# Autodesk Inventor assembly: mg996r leg bottom middle
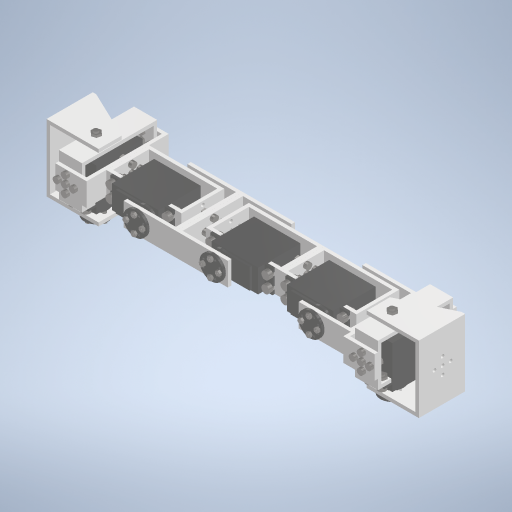
[picture p0: Inventor's stored thumbnail of the model, 512x512]
Saved by Autodesk Inventor 2023 (Build 270158000, 158)
## iProperties
Created: 2022-06-29
Part Number: mg996r leg bottom middle
Document SubType Name: Assembly
Designer: isamu
Author: isamu
## Documents named in this file (6)
- D:\personal_projects\robot\inventor\mg996r left leg bottom middle.iam
- D:\personal_projects\robot\inventor\mg996r 3mm middle base leg.iam
- D:\personal_projects\robot\inventor\mg996r 3mm foot.iam
- D:\personal_projects\robot\exports\frames\m3x8.ipt
- D:\personal_projects\robot\exports\frames\m3 nuts.ipt
- D:\personal_projects\robot\inventor\mg996r 3mm center frame.iam
## Components (23 placed, 5 different names)
1. mg996r 3mm middle base leg:1 [sub-assembly] — Mate:1, Mate:2, Mate:3, Insert:1, Insert:2, Insert:3, Insert:4, Insert:5, Mate:4, Mate:5, Mate:6, Insert:11, Insert:12, Insert:13, Insert:14, Insert:15
2. mg996r 3mm foot:1 [sub-assembly] — Mate:1, Mate:2, Mate:3, Insert:6, Insert:7, Insert:8, Insert:9, Insert:10
3. m3x8:1 — Insert:3
4. m3x8:2 — Insert:4
5. m3x8:3 — Insert:1
6. m3x8:4 — Insert:2
7. m3x8:5 — Insert:5
8. m3 nuts:1 — Insert:8
9. m3 nuts:2 — Insert:6
10. m3 nuts:3 — Insert:7
11. m3 nuts:4 — Insert:9
12. m3 nuts:5 — Insert:10
13. mg996r 3mm center frame:1 [sub-assembly] — Mate:4, Mate:5, Mate:6, Insert:16, Insert:17, Insert:18, Insert:19, Insert:20
14. m3 nuts:6 — Insert:17
15. m3 nuts:7 — Insert:20
16. m3 nuts:8 — Insert:16
17. m3 nuts:9 — Insert:19
18. m3 nuts:10 — Insert:18
19. m3x8:6 — Insert:15
20. m3x8:7 — Insert:13
21. m3x8:8 — Insert:12
22. m3x8:9 — Insert:14
23. m3x8:10 — Insert:11
## Relationships (26: Insert 20, Mate 6)
- Mate:1: mg996r 3mm middle base leg:1 ↔ mg996r 3mm foot:1
- Mate:2: mg996r 3mm middle base leg:1 ↔ mg996r 3mm foot:1
- Mate:3: mg996r 3mm middle base leg:1 ↔ mg996r 3mm foot:1
- Insert:1: mg996r 3mm middle base leg:1 ↔ m3x8:3
- Insert:2: mg996r 3mm middle base leg:1 ↔ m3x8:4
- Insert:3: mg996r 3mm middle base leg:1 ↔ m3x8:1
- Insert:4: mg996r 3mm middle base leg:1 ↔ m3x8:2
- Insert:5: mg996r 3mm middle base leg:1 ↔ m3x8:5
- Insert:6: mg996r 3mm foot:1 ↔ m3 nuts:2
- Insert:7: mg996r 3mm foot:1 ↔ m3 nuts:3
- Insert:8: mg996r 3mm foot:1 ↔ m3 nuts:1
- Insert:9: mg996r 3mm foot:1 ↔ m3 nuts:4
- Insert:10: mg996r 3mm foot:1 ↔ m3 nuts:5
- Mate:4: mg996r 3mm middle base leg:1 ↔ mg996r 3mm center frame:1
- Mate:5: mg996r 3mm middle base leg:1 ↔ mg996r 3mm center frame:1
- Mate:6: mg996r 3mm middle base leg:1 ↔ mg996r 3mm center frame:1
- Insert:11: mg996r 3mm middle base leg:1 ↔ m3x8:10
- Insert:12: mg996r 3mm middle base leg:1 ↔ m3x8:8
- Insert:13: mg996r 3mm middle base leg:1 ↔ m3x8:7
- Insert:14: mg996r 3mm middle base leg:1 ↔ m3x8:9
- Insert:15: mg996r 3mm middle base leg:1 ↔ m3x8:6
- Insert:16: mg996r 3mm center frame:1 ↔ m3 nuts:8
- Insert:17: mg996r 3mm center frame:1 ↔ m3 nuts:6
- Insert:18: mg996r 3mm center frame:1 ↔ m3 nuts:10
- Insert:19: mg996r 3mm center frame:1 ↔ m3 nuts:9
- Insert:20: mg996r 3mm center frame:1 ↔ m3 nuts:7
